# Autodesk Inventor assembly: axis_2_bottom_L_frame(bottom)
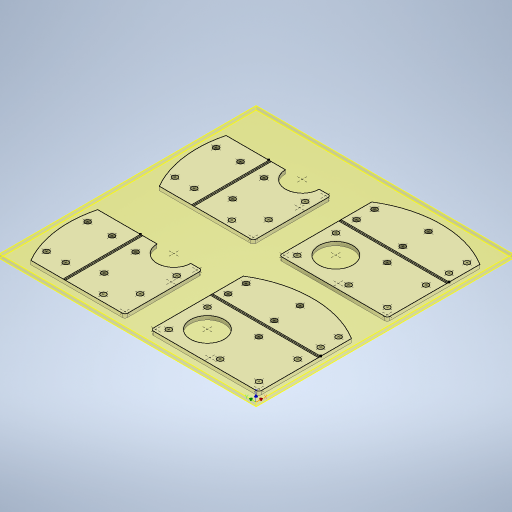
[picture p0: Inventor's stored thumbnail of the model, 512x512]
Saved by Autodesk Inventor 2024.2 (Build 282272000, 272)
## iProperties
Created: 2024-01-11
Part Number: axis_2_bottom_L_frame(bottom)
Document SubType Name: Assembly
Designer: chanh
Author: chanh
## Documents named in this file (3)
- C:\Users\chanh\내 드라이브\로봇\Humanoid\Roboin Humanoid Project\Inventor\rh_plus_7_axis_robot_arm_hardware\CAM\1.5T\new_L_frame\new_L_frame.iam
- C:\Users\chanh\내 드라이브\로봇\Humanoid\Roboin Humanoid Project\Inventor\rh_plus_7_axis_robot_arm_hardware\CAM\1.5T\new_L_frame\axis_2_bottom_L_frame(bottom).ipt
- C:\Users\chanh\내 드라이브\로봇\Humanoid\Roboin Humanoid Project\Inventor\rh_plus_7_axis_robot_arm_hardware\CAM\1.5T\new_L_frame\axis_2_bottom_L_frame(top).ipt
## Components (4 placed, 2 different names)
1. axis_2_bottom_L_frame(bottom):1 — Mate:1, Flush:1, Flush:2, Mate:2, Flush:3, Flush:4, Flush:7, Flush:8, Flush:9
2. axis_2_bottom_L_frame(top):1 — Mate:2, Flush:3, Flush:4
3. axis_2_bottom_L_frame(bottom):2 — Flush:7, Flush:8, Flush:9
4. axis_2_bottom_L_frame(top):2
## Relationships (12: Flush 9, Mate 3)
- Mate:1: axis_2_bottom_L_frame(bottom):1
- Flush:1: axis_2_bottom_L_frame(bottom):1
- Flush:2: axis_2_bottom_L_frame(bottom):1
- Mate:2 (10 mm): axis_2_bottom_L_frame(bottom):1 ↔ axis_2_bottom_L_frame(top):1
- Flush:3: axis_2_bottom_L_frame(bottom):1 ↔ axis_2_bottom_L_frame(top):1
- Flush:4: axis_2_bottom_L_frame(bottom):1 ↔ axis_2_bottom_L_frame(top):1
- [Mate] (10 mm): axis_2_bottom_L_frame(bottom):2 ↔ axis_2_bottom_L_frame(top):2
- [Flush]: axis_2_bottom_L_frame(bottom):2 ↔ axis_2_bottom_L_frame(top):2
- [Flush]: axis_2_bottom_L_frame(bottom):2 ↔ axis_2_bottom_L_frame(top):2
- Flush:7 (-50 mm): axis_2_bottom_L_frame(bottom):1 ↔ axis_2_bottom_L_frame(bottom):2
- Flush:8: axis_2_bottom_L_frame(bottom):1 ↔ axis_2_bottom_L_frame(bottom):2
- Flush:9: axis_2_bottom_L_frame(bottom):1 ↔ axis_2_bottom_L_frame(bottom):2
## Named parameters: d6_d3 = 10 mm, d7_d4 = 0 mm, d8_d5 = 0 mm
